# Autodesk Inventor assembly: BeamcBenchAdjustable
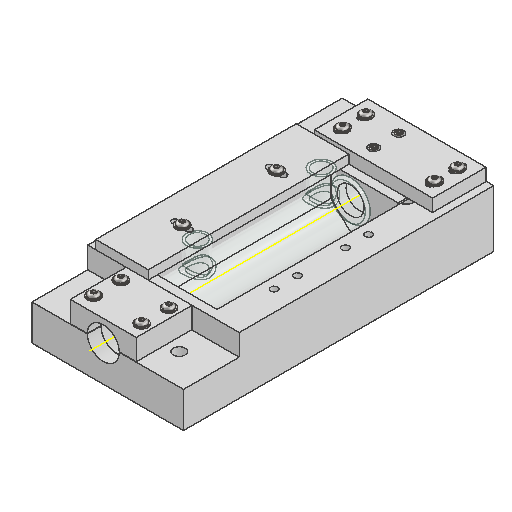
[picture p0: Inventor's stored thumbnail of the model, 512x512]
Saved by Autodesk Inventor 2025.1 (Build 291241020, 241B)
## iProperties
Created: 2024-09-23
Part Number: BeamcBenchAdjustable
Document SubType Name: Assembly
Designer: wayneslade
Author: wayneslade
## Documents named in this file (18)
- C:\Users\wayneslade\OneDrive - OceanSense, LLC\Documents\Inventor\BeamcBench\BeamcBenchAdjustable.iam
- C:\Users\wayneslade\OneDrive - OceanSense, LLC\Documents\Inventor\BeamcBench\Cuvette Holder Adjustable Trans.ipt
- C:\Users\wayneslade\OneDrive - OceanSense, LLC\Documents\Inventor\BeamcBench\Cuvette10mm.ipt
- C:\Users\wayneslade\OneDrive - OceanSense, LLC\Documents\Inventor\BeamcBench\Cuvette Holder Adjustable Recv.ipt
- C:\Users\wayneslade\OneDrive - OceanSense, LLC\Documents\Inventor\BeamcBench\Cuvette Holder Transmit Holddown.ipt
- C:\Users\wayneslade\OneDrive - OceanSense, LLC\Documents\Inventor\BeamcBench\Cuvette50mmFisher.ipt
- C:\Users\wayneslade\OneDrive - OceanSense, LLC\Documents\Inventor\BeamcBench\Cuvette Aligner 50mm.ipt
- C:\Users\wayneslade\OneDrive - OceanSense, LLC\Documents\Inventor\BeamcBench\Cuvette Aligner 10mm.ipt
- C:\Users\wayneslade\OneDrive - OceanSense, LLC\Documents\Inventor\BeamcBench\Cuvette100mmStarna.ipt
- C:\Users\wayneslade\OneDrive - OceanSense, LLC\Documents\Inventor\BeamcBench\Cuvette Aligner 100mmStarna.ipt
- C:\Users\wayneslade\OneDrive - OceanSense, LLC\Documents\Inventor\BeamcBench\Cuvette Aligner 100mm Flat Edge.ipt
- C:\Users\wayneslade\OneDrive - OceanSense, LLC\Documents\Inventor\HardwareComponents\Ruthex Inserts\ruthex RX-M3-5,7.ipt
- C:\Users\wayneslade\OneDrive - OceanSense, LLC\Documents\Inventor\HardwareComponents\Ruthex Inserts\ruthex RX-M4x8.1.ipt
- C:\Users\wayneslade\OneDrive - OceanSense, LLC\Documents\Inventor\Content Center Files\R2025\en-US\ISO 7089\ISO 7089 - 3 - 140 HV(1).ipt
- C:\Users\wayneslade\OneDrive - OceanSense, LLC\Documents\Inventor\Content Center Files\R2025\en-US\ISO 7380-1\ISO 7380-1 - M3 x 12.ipt
- C:\Users\wayneslade\OneDrive - OceanSense, LLC\Documents\Inventor\Content Center Files\R2025\en-US\AS 1421(2)\AS 1421 - M4 x 10 Cup Point.ipt
- C:\Users\wayneslade\OneDrive - OceanSense, LLC\Documents\Inventor\Content Center Files\R2025\en-US\ISO 7380-1\ISO 7380-1 - M3 x 10.ipt
- C:\Users\wayneslade\OneDrive - OceanSense, LLC\Documents\Inventor\Content Center Files\R2025\en-US\ISO 7380-1\ISO 7380-1 - M3 x 20.ipt
## Components (53 placed, 17 different names)
1. Cuvette Holder Adjustable Trans:1 — Mate:1, Mate:2, Flush:1, Flush:2, Flush:3, Flush:6, Flush:7, Mate:4, Mate:7, Mate:8, Flush:8, Flush:9, Mate:10, Mate:11, Flush:10, Flush:11, Mate:12, Angle:3, Flush:12, Flush:13, Flush:15, Mate:15, Mate:16, Mate:17, Mate:18, Mate:19, Mate:20, Mate:21, Mate:22, Mate:23, Mate:24, Mate:25, Mate:26, Mate:27, Mate:28, Mate:29, Mate:30, Mate:31, Mate:32, Mate:35, Mate:37, Mate:55, Mate:57, Mate:62, Mate:64
2. Cuvette10mm:1 — Mate:2, Mate:3, Angle:1, Mate:9
3. Cuvette Holder Adjustable Recv:1 — Flush:4, Flush:5, Mate:33, Mate:34, Mate:36, Mate:38, Mate:56, Mate:58
4. Cuvette Holder Transmit Holddown:1 — Flush:6, Flush:7, Mate:65, Mate:66, Mate:67, Mate:68, Mate:69, Mate:70, Mate:71, Mate:72
5. Cuvette50mmFisher:1 — Mate:4, Mate:5, Angle:2, Mate:6
6. Cuvette Holder Adjustable Recv:2 — Mate:6, Mate:7, Mate:8
7. Cuvette Aligner 50mmFisher:1 — Flush:8, Flush:9
8. Cuvette Holder Adjustable Recv:3 — Mate:9, Mate:10, Mate:11
9. Cuvette Aligner 10mm:1 — Flush:10, Flush:11
10. Cuvette100mmStarna:1 — Mate:12, Mate:13, Angle:3, Tangent:1
11. Cuvette Aligner 100mmStarna — Flush:12, Flush:13
12. Cuvette Aligner 100mm Flat Edge:1 — Flush:15, Mate:15, Tangent:1, Mate:61, Mate:63
13. ruthex RX-M4x8.1:1 — Mate:33, Mate:60
14. ruthex RX-M4x8.1:2 — Mate:34, Mate:59
15. ruthex RX-M3-5,7:1 — Mate:16
16. ruthex RX-M3-5,7:2 — Mate:17
17. ruthex RX-M3-5,7:3 — Mate:18
18. ruthex RX-M3-5,7:4 — Mate:19
19. ruthex RX-M3-5,7:5 — Mate:20
20. ruthex RX-M3-5,7:6 — Mate:21
21. ruthex RX-M3-5,7:7 — Mate:23
22. ruthex RX-M3-5,7:8 — Mate:22
23. ruthex RX-M3-5,7:9 — Mate:28
24. ruthex RX-M3-5,7:10 — Mate:27
25. ruthex RX-M3-5,7:11 — Mate:26
26. ruthex RX-M3-5,7:12 — Mate:25
27. ruthex RX-M3-5,7:13 — Mate:24
28. ruthex RX-M3-5,7:14 — Mate:31
29. ruthex RX-M3-5,7:15 — Mate:30
30. ruthex RX-M3-5,7:16 — Mate:32
31. ruthex RX-M3-5,7:17 — Mate:29
32. ISO 7089 3:1 — Mate:35, Mate:36, Insert:1
33. ISO 7380-1 M3 x 12:1 — Insert:1
34. ISO 7089 3:2 — Mate:37, Mate:38, Insert:2
35. ISO 7089 3:11 — Mate:55, Mate:56, Insert:11
36. ISO 7089 3:12 — Mate:57, Mate:58, Insert:12
37. ISO 7380-1 M3 x 12:2 — Insert:2
38. ISO 7380-1 M3 x 12:11 — Insert:11
39. ISO 7380-1 M3 x 12:12 — Insert:12
40. AS 1421 Cup Point - Metric M4 x 10 Cup Point:1 — Mate:60
41. AS 1421 Cup Point - Metric M4 x 10 Cup Point:2 — Mate:59
42. ISO 7089 3:13 — Mate:61
43. ISO 7380-1 M3 x 10:1 — Mate:62
44. ISO 7089 3:14 — Mate:63
45. ISO 7380-1 M3 x 10:2 — Mate:64
46. ISO 7089 3:15 — Mate:65, Mate:66, Insert:15
47. ISO 7380-1 M3 x 20:1 — Insert:15
48. ISO 7089 3:16 — Mate:67, Mate:68, Insert:16
49. ISO 7089 3:17 — Mate:69, Mate:70, Insert:17
50. ISO 7089 3:18 — Mate:71, Mate:72, Insert:18
51. ISO 7380-1 M3 x 20:2 — Insert:16
52. ISO 7380-1 M3 x 20:3 — Insert:17
53. ISO 7380-1 M3 x 20:4 — Insert:18
## Relationships (83: Mate 55, Flush 14, Insert 10, Angle 3, Tangent 1)
- Mate:1: Cuvette Holder Adjustable Trans:1
- Mate:2: Cuvette Holder Adjustable Trans:1 ↔ Cuvette10mm:1
- Mate:3: Cuvette10mm:1
- Angle:1 (0 deg): Cuvette10mm:1
- Flush:1 (12.5 mm): Cuvette Holder Adjustable Trans:1
- Flush:2 (52.5 mm): Cuvette Holder Adjustable Trans:1
- Flush:3 (102.5 mm): Cuvette Holder Adjustable Trans:1
- Flush:4: Cuvette Holder Adjustable Recv:1
- Flush:5: Cuvette Holder Adjustable Recv:1
- Flush:6: Cuvette Holder Adjustable Trans:1 ↔ Cuvette Holder Transmit Holddown:1
- Flush:7: Cuvette Holder Adjustable Trans:1 ↔ Cuvette Holder Transmit Holddown:1
- Mate:4: Cuvette Holder Adjustable Trans:1 ↔ Cuvette50mmFisher:1
- Mate:5: Cuvette50mmFisher:1
- Angle:2 (-90 deg): Cuvette50mmFisher:1
- Mate:6: Cuvette50mmFisher:1 ↔ Cuvette Holder Adjustable Recv:2
- Mate:7: Cuvette Holder Adjustable Trans:1 ↔ Cuvette Holder Adjustable Recv:2
- Mate:8: Cuvette Holder Adjustable Trans:1 ↔ Cuvette Holder Adjustable Recv:2
- Flush:8: Cuvette Holder Adjustable Trans:1 ↔ Cuvette Aligner 50mmFisher:1
- Flush:9: Cuvette Holder Adjustable Trans:1 ↔ Cuvette Aligner 50mmFisher:1
- Mate:9: Cuvette10mm:1 ↔ Cuvette Holder Adjustable Recv:3
- Mate:10: Cuvette Holder Adjustable Trans:1 ↔ Cuvette Holder Adjustable Recv:3
- Mate:11: Cuvette Holder Adjustable Trans:1 ↔ Cuvette Holder Adjustable Recv:3
- Flush:10: Cuvette Holder Adjustable Trans:1 ↔ Cuvette Aligner 10mm:1
- Flush:11: Cuvette Holder Adjustable Trans:1 ↔ Cuvette Aligner 10mm:1
- Mate:12: Cuvette Holder Adjustable Trans:1 ↔ Cuvette100mmStarna:1
- Mate:13: Cuvette100mmStarna:1
- Angle:3 (-90 deg): Cuvette Holder Adjustable Trans:1 ↔ Cuvette100mmStarna:1
- Flush:12: Cuvette Holder Adjustable Trans:1 ↔ Cuvette Aligner 100mmStarna
- Flush:13: Cuvette Holder Adjustable Trans:1 ↔ Cuvette Aligner 100mmStarna
- Flush:15: Cuvette Holder Adjustable Trans:1 ↔ Cuvette Aligner 100mm Flat Edge:1
- Mate:15: Cuvette Holder Adjustable Trans:1 ↔ Cuvette Aligner 100mm Flat Edge:1
- Tangent:1: Cuvette100mmStarna:1 ↔ Cuvette Aligner 100mm Flat Edge:1
- Mate:16: Cuvette Holder Adjustable Trans:1 ↔ ruthex RX-M3-5,7:1
- Mate:17: Cuvette Holder Adjustable Trans:1 ↔ ruthex RX-M3-5,7:2
- Mate:18: Cuvette Holder Adjustable Trans:1 ↔ ruthex RX-M3-5,7:3
- Mate:19: Cuvette Holder Adjustable Trans:1 ↔ ruthex RX-M3-5,7:4
- Mate:20: Cuvette Holder Adjustable Trans:1 ↔ ruthex RX-M3-5,7:5
- Mate:21: Cuvette Holder Adjustable Trans:1 ↔ ruthex RX-M3-5,7:6
- Mate:22: Cuvette Holder Adjustable Trans:1 ↔ ruthex RX-M3-5,7:8
- Mate:23: Cuvette Holder Adjustable Trans:1 ↔ ruthex RX-M3-5,7:7
- Mate:24: Cuvette Holder Adjustable Trans:1 ↔ ruthex RX-M3-5,7:13
- Mate:25: Cuvette Holder Adjustable Trans:1 ↔ ruthex RX-M3-5,7:12
- Mate:26: Cuvette Holder Adjustable Trans:1 ↔ ruthex RX-M3-5,7:11
- Mate:27: Cuvette Holder Adjustable Trans:1 ↔ ruthex RX-M3-5,7:10
- Mate:28: Cuvette Holder Adjustable Trans:1 ↔ ruthex RX-M3-5,7:9
- Mate:29: Cuvette Holder Adjustable Trans:1 ↔ ruthex RX-M3-5,7:17
- Mate:30: Cuvette Holder Adjustable Trans:1 ↔ ruthex RX-M3-5,7:15
- Mate:31: Cuvette Holder Adjustable Trans:1 ↔ ruthex RX-M3-5,7:14
- Mate:32: Cuvette Holder Adjustable Trans:1 ↔ ruthex RX-M3-5,7:16
- Mate:33: Cuvette Holder Adjustable Recv:1 ↔ ruthex RX-M4x8.1:1
- Mate:34: Cuvette Holder Adjustable Recv:1 ↔ ruthex RX-M4x8.1:2
- Mate:35: Cuvette Holder Adjustable Trans:1 ↔ ISO 7089 3:1
- Mate:36: Cuvette Holder Adjustable Recv:1 ↔ ISO 7089 3:1
- Mate:37: Cuvette Holder Adjustable Trans:1 ↔ ISO 7089 3:2
- Mate:38: Cuvette Holder Adjustable Recv:1 ↔ ISO 7089 3:2
- Mate:55: Cuvette Holder Adjustable Trans:1 ↔ ISO 7089 3:11
- Mate:56: Cuvette Holder Adjustable Recv:1 ↔ ISO 7089 3:11
- Mate:57: Cuvette Holder Adjustable Trans:1 ↔ ISO 7089 3:12
- Mate:58: Cuvette Holder Adjustable Recv:1 ↔ ISO 7089 3:12
- Insert:1: ISO 7089 3:1 ↔ ISO 7380-1 M3 x 12:1
- Insert:2: ISO 7089 3:2 ↔ ISO 7380-1 M3 x 12:2
- Insert:11: ISO 7089 3:11 ↔ ISO 7380-1 M3 x 12:11
- Insert:12: ISO 7089 3:12 ↔ ISO 7380-1 M3 x 12:12
- Mate:59: ruthex RX-M4x8.1:2 ↔ AS 1421 Cup Point - Metric M4 x 10 Cup Point:2
- Mate:60: ruthex RX-M4x8.1:1 ↔ AS 1421 Cup Point - Metric M4 x 10 Cup Point:1
- [Insert]: ISO 7089 3:13 ↔ ISO 7380-1 M3 x 10:1
- Mate:61: Cuvette Aligner 100mm Flat Edge:1 ↔ ISO 7089 3:13
- Mate:62: Cuvette Holder Adjustable Trans:1 ↔ ISO 7380-1 M3 x 10:1
- [Insert]: ISO 7089 3:14 ↔ ISO 7380-1 M3 x 10:2
- Mate:63: Cuvette Aligner 100mm Flat Edge:1 ↔ ISO 7089 3:14
- Mate:64: Cuvette Holder Adjustable Trans:1 ↔ ISO 7380-1 M3 x 10:2
- Mate:65: Cuvette Holder Transmit Holddown:1 ↔ ISO 7089 3:15
- Mate:66: Cuvette Holder Transmit Holddown:1 ↔ ISO 7089 3:15
- Mate:67: Cuvette Holder Transmit Holddown:1 ↔ ISO 7089 3:16
- Mate:68: Cuvette Holder Transmit Holddown:1 ↔ ISO 7089 3:16
- Mate:69: Cuvette Holder Transmit Holddown:1 ↔ ISO 7089 3:17
- Mate:70: Cuvette Holder Transmit Holddown:1 ↔ ISO 7089 3:17
- Mate:71: Cuvette Holder Transmit Holddown:1 ↔ ISO 7089 3:18
- Mate:72: Cuvette Holder Transmit Holddown:1 ↔ ISO 7089 3:18
- Insert:15: ISO 7089 3:15 ↔ ISO 7380-1 M3 x 20:1
- Insert:16: ISO 7089 3:16 ↔ ISO 7380-1 M3 x 20:2
- Insert:17: ISO 7089 3:17 ↔ ISO 7380-1 M3 x 20:3
- Insert:18: ISO 7089 3:18 ↔ ISO 7380-1 M3 x 20:4
## Named parameters: d127_d86 = 0 mm, d128_d87 = 0 mm, d129_d88 = 0 mm, d132_d127_d86 = 0 mm, d133_d128_d87 = 0 mm, d134_d129_d88 = 0 mm
